# Autodesk Inventor assembly: Final assembly 2
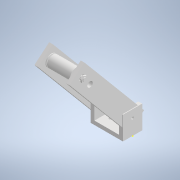
[picture p0: Inventor's stored thumbnail of the model, 180x180]
Saved by Autodesk Inventor 2022 (Build 260153000, 153)
## iProperties
Created: 2022-06-16
Part Number: Final assembly 2
Document SubType Name: Assembly
Designer: chait
Author: chait
## Documents named in this file (3)
- C:\Users\chait\Documents\Final assembly 2.iam
- C:\Users\chait\Documents\clamp.ipt
- C:\Users\chait\Documents\final assembly 1.iam
## Components (2 placed, 2 different names)
1. clamp:1 — Insert:1, Angle:1, Angle:2
2. final assembly 1:1 [sub-assembly] — Insert:1, Angle:1, Angle:2
## Relationships (3: Angle 2, Insert 1)
- Insert:1: clamp:1 ↔ final assembly 1:1
- Angle:1 (45 deg): clamp:1 ↔ final assembly 1:1
- Angle:2 (50 deg): clamp:1 ↔ final assembly 1:1
